# Autodesk Inventor assembly: Electronics_assembly
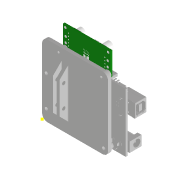
[picture p0: Inventor's stored thumbnail of the model, 180x180]
Saved by Autodesk Inventor 2022 (Build 260153000, 153)
## iProperties
Created: 2022-09-21
Part Number: Electronics_assembly
Document SubType Name: Assembly
Designer: dell
Author: dell
## Documents named in this file (4)
- D:\xxxx\Uni\Part IV\MECHENG_700\Part_IV_project_CAD\Bird_skeleton_prototypes\Wing_drone_V1\Electronics\Electronics_assembly.iam
- D:\xxxx\Uni\Part IV\MECHENG_700\Part_IV_project_CAD\Bird_skeleton_prototypes\Wing_drone_V1\Electronics\Electronics_mount.ipt
- D:\xxxx\Uni\Part IV\MECHENG_700\Part_IV_project_CAD\Bird_skeleton_prototypes\Wing_drone_V1\Electronics\Arduino_uno.iam
- D:\xxxx\Uni\Part IV\MECHENG_700\Part_IV_project_CAD\Bird_skeleton_prototypes\Wing_drone_V1\Electronics\s18v20x_voltage-regulator.ipt
## Components (3 placed, 3 different names)
1. Electronics_mount:2 — Mate:1, Mate:2, Mate:3, Mate:4, Mate:5, Mate:6
2. Arduino_uno:1 [sub-assembly] — Mate:1, Mate:2, Mate:3
3. s18v20x_voltage-regulator:2 — Mate:4, Mate:5, Mate:6
## Relationships (6: Mate 6)
- Mate:1: Electronics_mount:2 ↔ Arduino_uno:1
- Mate:2: Electronics_mount:2 ↔ Arduino_uno:1
- Mate:3: Electronics_mount:2 ↔ Arduino_uno:1
- Mate:4: Electronics_mount:2 ↔ s18v20x_voltage-regulator:2
- Mate:5: Electronics_mount:2 ↔ s18v20x_voltage-regulator:2
- Mate:6: Electronics_mount:2 ↔ s18v20x_voltage-regulator:2
